# Autodesk Inventor assembly: ZB-Füllstandsmessung
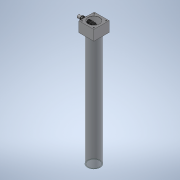
[picture p0: Inventor's stored thumbnail of the model, 180x180]
Saved by Autodesk Inventor 2021 (Build 250183000, 183)
## iProperties
Created: 2021-04-27
Part Number: ZB-Füllstandsmessung
Material: Generisch
Document SubType Name: Assembly
Designer: Michael
Author: Michael
## Documents named in this file (3)
- C:\Users\Sebastian Seewald\Documents\Inventor\Konstruktion_Studium\Lernfabrik\104_Extrudereinheit\204.002.01_ZB_Fuehlstandsmessung.iam
- C:\Users\Sebastian Seewald\Documents\Inventor\Konstruktion_Studium\Lernfabrik\104_Extrudereinheit\204.001.01_ZB_Sensor_Aufnahme.iam
- C:\Users\Sebastian Seewald\Documents\Inventor\Konstruktion_Studium\Lernfabrik\104_Extrudereinheit\504.005.01_Plexiglas_Rohr.ipt
## Components (2 placed, 2 different names)
1. 504.005.01_Plexiglas_Rohr:1 — Passend:3, Passend:4
2. 204.001.01_ZB_Sensor_Aufnahme:1 [sub-assembly] — Passend:1, Passend:2, Passend:3, Passend:4
## Relationships (4: Mate 4)
- Passend:1 [Mate]: 204.001.01_ZB_Sensor_Aufnahme:1
- Passend:2 [Mate]: 204.001.01_ZB_Sensor_Aufnahme:1
- Passend:3 [Mate]: 504.005.01_Plexiglas_Rohr:1 ↔ 204.001.01_ZB_Sensor_Aufnahme:1
- Passend:4 [Mate]: 504.005.01_Plexiglas_Rohr:1 ↔ 204.001.01_ZB_Sensor_Aufnahme:1
